# Autodesk Inventor assembly: Toggle Push Clamp
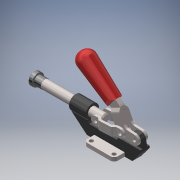
[picture p0: Inventor's stored thumbnail of the model, 180x180]
Saved by Autodesk Inventor 2019 (Build 230136000, 136)
## iProperties
Created: 2017-12-03
Part Number: Toggle Push Clamp
Document SubType Name: Assembly
Designer: maste
Author: maste
Sending System: SolidWorks 2017
Last Author: Radek Neckař
Last Saved: 2017-12-03
## Documents named in this file (8)
- D:\Summer Drive Base V1\Summer Drivebase\Toggle Push Clamp.iam
- D:\Summer Drive Base V1\Summer Drivebase\Part1.ipt
- D:\Summer Drive Base V1\Summer Drivebase\Part6.ipt
- D:\Summer Drive Base V1\Summer Drivebase\Part2.ipt
- D:\Summer Drive Base V1\Summer Drivebase\Part5.ipt
- D:\Summer Drive Base V1\Summer Drivebase\Part3.ipt
- D:\Summer Drive Base V1\Summer Drivebase\Part7.ipt
- D:\Summer Drive Base V1\Summer Drivebase\Part4.ipt
## Components (8 placed, 7 different names)
1. Part1:1 — Mate:3, Mate:13, Mate:14, Mate:16, Mate:17, Flush:1
2. Part6:1 — Mate:16, Mate:17, Flush:1
3. Part2:1 — Mate:5, Mate:6, Mate:7, Mate:8, Mate:9, Mate:10, Mate:11, Mate:12, Mate:13, Mate:14
4. Part5:1 — Mate:1, Mate:2, Rotation:1, Mate:3, Mate:4, Mate:15
5. Part3:1 — Mate:4, Mate:5, Mate:6
6. Part3:2 — Mate:7, Mate:8, Mate:15
7. Part7:1 — Mate:1, Mate:2, Rotation:1
8. Part4:1 — Mate:9, Mate:10, Mate:11, Mate:12
## Relationships (19: Mate 17, RelateRotation 1, Flush 1)
- Mate:1: Part5:1 ↔ Part7:1
- Mate:2: Part5:1 ↔ Part7:1
- Rotation:1 [RelateRotation] (1 ul): Part5:1 ↔ Part7:1
- Mate:3: Part1:1 ↔ Part5:1
- Mate:4: Part5:1 ↔ Part3:1
- Mate:5: Part2:1 ↔ Part3:1
- Mate:6: Part2:1 ↔ Part3:1
- Mate:7: Part2:1 ↔ Part3:2
- Mate:8: Part2:1 ↔ Part3:2
- Mate:9: Part2:1 ↔ Part4:1
- Mate:10: Part2:1 ↔ Part4:1
- Mate:11: Part2:1 ↔ Part4:1
- Mate:12: Part2:1 ↔ Part4:1
- Mate:13: Part1:1 ↔ Part2:1
- Mate:14: Part1:1 ↔ Part2:1
- Mate:15: Part5:1 ↔ Part3:2
- Mate:16: Part1:1 ↔ Part6:1
- Mate:17: Part1:1 ↔ Part6:1
- Flush:1 (-14 mm): Part1:1 ↔ Part6:1
